# Autodesk Inventor assembly: inner_glide_carriage_with_roller_assembly
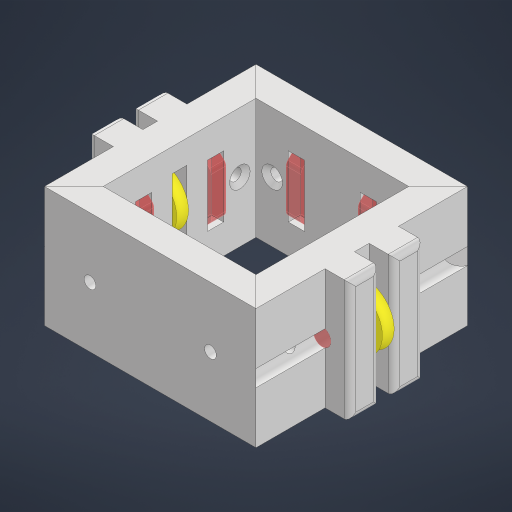
[picture p0: Inventor's stored thumbnail of the model, 512x512]
Saved by Autodesk Inventor 2024 (Build 280153000, 153)
## iProperties
Created: 2023-05-24
Part Number: inner_glide_carriage_with_roller_assembly
Document SubType Name: Assembly
Designer: aasmu
Author: aasmu
## Documents named in this file (7)
- C:\Users\aasmu\Documents\standing_desk\inner_glide_carriage_with_roller_assembly.iam
- C:\Users\aasmu\Documents\standing_desk\3_inner_glider_carriage_one_side.ipt
- C:\Users\aasmu\Documents\standing_desk\5_inner_glide_carraige_one_side_with_cabel_roller.ipt
- C:\Users\aasmu\Documents\standing_desk\steal_glide_plate.ipt
- C:\Users\aasmu\Documents\standing_desk\load_bearing.ipt
- C:\Users\aasmu\Documents\standing_desk\roller_shaft.ipt
- C:\Users\aasmu\Documents\standing_desk\cable_roller.ipt
## Components (20 placed, 6 different names)
1. 3_inner_glider_carriage_one_side:1 — Rigid:1, Rigid:2, Rigid:4, Rigid:5
2. 3_inner_glider_carriage_one_side:2 — Rigid:3, Rigid:8, Rigid:9
3. 5_inner_glide_carraige_one_side_with_cabel_roller:1 — Rigid:2, Rigid:6, Rigid:7, Rotational:3, Rigid:12, Rigid:13
4. 5_inner_glide_carraige_one_side_with_cabel_roller:2 — Rigid:1, Rigid:3, Rigid:10, Rigid:11, Rigid:14, Rigid:15, Rigid:16
5. steal_glide_plate:1 — Rigid:5
6. steal_glide_plate:2 — Rigid:4
7. steal_glide_plate:3 — Rigid:7
8. steal_glide_plate:4 — Rigid:6
9. steal_glide_plate:5 — Rigid:8
10. steal_glide_plate:6 — Rigid:9
11. steal_glide_plate:7 — Rigid:10
12. steal_glide_plate:8 — Rigid:11
13. load_bearing:1 — Rotational:3
14. load_bearing:2 — Rigid:12
15. load_bearing:3 — Rigid:15
16. load_bearing:4 — Rigid:14
17. roller_shaft:1 — Rotational:1, Rigid:16
18. roller_shaft:2 — Rotational:2, Rigid:13
19. cable_roller:1 — Rotational:1
20. cable_roller:2 — Rotational:2
## Relationships (19: WeldJoint 16, RevoluteJoint 3)
- Rigid:1 [WeldJoint]: 3_inner_glider_carriage_one_side:1 ↔ 5_inner_glide_carraige_one_side_with_cabel_roller:2
- Rigid:2 [WeldJoint]: 3_inner_glider_carriage_one_side:1 ↔ 5_inner_glide_carraige_one_side_with_cabel_roller:1
- Rigid:3 [WeldJoint]: 3_inner_glider_carriage_one_side:2 ↔ 5_inner_glide_carraige_one_side_with_cabel_roller:2
- Rigid:4 [WeldJoint]: 3_inner_glider_carriage_one_side:1 ↔ steal_glide_plate:2
- Rigid:5 [WeldJoint]: 3_inner_glider_carriage_one_side:1 ↔ steal_glide_plate:1
- Rigid:6 [WeldJoint]: 5_inner_glide_carraige_one_side_with_cabel_roller:1 ↔ steal_glide_plate:4
- Rigid:7 [WeldJoint]: 5_inner_glide_carraige_one_side_with_cabel_roller:1 ↔ steal_glide_plate:3
- Rigid:8 [WeldJoint]: 3_inner_glider_carriage_one_side:2 ↔ steal_glide_plate:5
- Rigid:9 [WeldJoint]: 3_inner_glider_carriage_one_side:2 ↔ steal_glide_plate:6
- Rigid:10 [WeldJoint]: 5_inner_glide_carraige_one_side_with_cabel_roller:2 ↔ steal_glide_plate:7
- Rigid:11 [WeldJoint]: 5_inner_glide_carraige_one_side_with_cabel_roller:2 ↔ steal_glide_plate:8
- Rotational:1 [RevoluteJoint]: roller_shaft:1 ↔ cable_roller:1
- Rotational:2 [RevoluteJoint]: roller_shaft:2 ↔ cable_roller:2
- Rotational:3 [RevoluteJoint]: 5_inner_glide_carraige_one_side_with_cabel_roller:1 ↔ load_bearing:1
- Rigid:12 [WeldJoint]: 5_inner_glide_carraige_one_side_with_cabel_roller:1 ↔ load_bearing:2
- Rigid:13 [WeldJoint]: 5_inner_glide_carraige_one_side_with_cabel_roller:1 ↔ roller_shaft:2
- Rigid:14 [WeldJoint]: 5_inner_glide_carraige_one_side_with_cabel_roller:2 ↔ load_bearing:4
- Rigid:15 [WeldJoint]: 5_inner_glide_carraige_one_side_with_cabel_roller:2 ↔ load_bearing:3
- Rigid:16 [WeldJoint]: 5_inner_glide_carraige_one_side_with_cabel_roller:2 ↔ roller_shaft:1
